# Autodesk Inventor assembly: Pin, Arm 1 Assembly
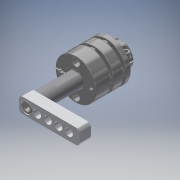
[picture p0: Inventor's stored thumbnail of the model, 180x180]
Saved by Autodesk Inventor 2016 (Build 200138000, 138)
## iProperties
Created: 2015-07-08
Part Number: Pin, Arm 1 Assembly
Document SubType Name: Assembly
Designer: Dennis
Author: Dennis
## Documents named in this file (5)
- C:\Users\Dennis\Dropbox\NI Work\NI Ball Bearing Slider Crank\CAD\Assemblies\Pin, Arm 1 Assembly.iam
- C:\Users\Dennis\Dropbox\NI Work\NI Ball Bearing Slider Crank\CAD\Arm 1.ipt
- C:\Users\Dennis\Dropbox\NI Work\NI Ball Bearing Slider Crank\CAD\McMaster Parts\.25-20x.5.ipt
- C:\Users\Dennis\Dropbox\NI Work\NI Ball Bearing Slider Crank\CAD\McMaster Parts\Coupling - Servomotor Flexible Shaft Coupling, 1_4 x 1_2 Shaft Diameter, 1.488 Length, 1.34 OD - 2764K312.ipt
- C:\Users\Dennis\Dropbox\NI Work\NI Ball Bearing Slider Crank\CAD\Pin V2.ipt
## Components (4 placed, 4 different names)
1. Arm 1:1 — Mate:4, Mate:9, Angle:3, Mate:12
2. .25-20x.5:1 — Mate:4, Mate:9, Mate:11
3. Coupling - Servomotor Flexible Shaft Coupling, 1_4 x 1_2 Shaft Diameter, 1.488 Length, 1.34 OD - 2764K312:1 — Angle:2, Angle:3, Mate:10, Flush:1
4. Pin V2:1 — Mate:10, Flush:1, Mate:11, Mate:12
## Relationships (8: Mate 5, Angle 2, Flush 1)
- Mate:4: Arm 1:1 ↔ .25-20x.5:1
- Mate:9: Arm 1:1 ↔ .25-20x.5:1
- Angle:2 (0 deg): Coupling - Servomotor Flexible Shaft Coupling, 1_4 x 1_2 Shaft Diameter, 1.488 Length, 1.34 OD - 2764K312:1
- Angle:3 (0 deg): Arm 1:1 ↔ Coupling - Servomotor Flexible Shaft Coupling, 1_4 x 1_2 Shaft Diameter, 1.488 Length, 1.34 OD - 2764K312:1
- Mate:10: Coupling - Servomotor Flexible Shaft Coupling, 1_4 x 1_2 Shaft Diameter, 1.488 Length, 1.34 OD - 2764K312:1 ↔ Pin V2:1
- Flush:1: Coupling - Servomotor Flexible Shaft Coupling, 1_4 x 1_2 Shaft Diameter, 1.488 Length, 1.34 OD - 2764K312:1 ↔ Pin V2:1
- Mate:11: .25-20x.5:1 ↔ Pin V2:1
- Mate:12: Arm 1:1 ↔ Pin V2:1
